# Autodesk Inventor assembly: Small-Servo-Holder
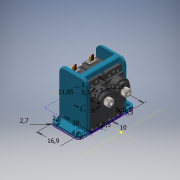
[picture p0: Inventor's stored thumbnail of the model, 180x180]
Saved by Autodesk Inventor 2018.2 (Build 222227000, 227)
## iProperties
Created: 2018-02-21
Part Number: Small-Servo-Holder
Material: Generisch
Document SubType Name: Assembly
Designer: JochenAlt
Author: JochenAlt
## Documents named in this file (3)
- D:\Projects\Donna\CAD\Small-Servo-Holder.iam
- D:\Projects\Donna\CAD\Stewart-Small-Servo-Holder.ipt
- D:\Projects\Donna\CAD\Hitec HS-5065MG.ipt
## Components (3 placed, 2 different names)
1. Stewart-Small-Servo-Holder:1 — Passend:1, Passend:2, Passend:3, Passend:4, Winkel:1, Winkel:2
2. Hitec HS-5065MG:1 — Passend:1, Passend:4, Winkel:1
3. Hitec HS-5065MG:2 — Passend:2, Passend:3, Winkel:2
## Relationships (6: Mate 4, Angle 2)
- Passend:1 [Mate]: Stewart-Small-Servo-Holder:1 ↔ Hitec HS-5065MG:1
- Passend:2 [Mate]: Stewart-Small-Servo-Holder:1 ↔ Hitec HS-5065MG:2
- Passend:3 [Mate] (0.3 mm): Stewart-Small-Servo-Holder:1 ↔ Hitec HS-5065MG:2
- Passend:4 [Mate] (0.3 mm): Stewart-Small-Servo-Holder:1 ↔ Hitec HS-5065MG:1
- Winkel:1 [Angle] (180 deg): Stewart-Small-Servo-Holder:1 ↔ Hitec HS-5065MG:1
- Winkel:2 [Angle] (180 deg): Stewart-Small-Servo-Holder:1 ↔ Hitec HS-5065MG:2
